# Autodesk Inventor assembly: ASY Рама №2 платформа
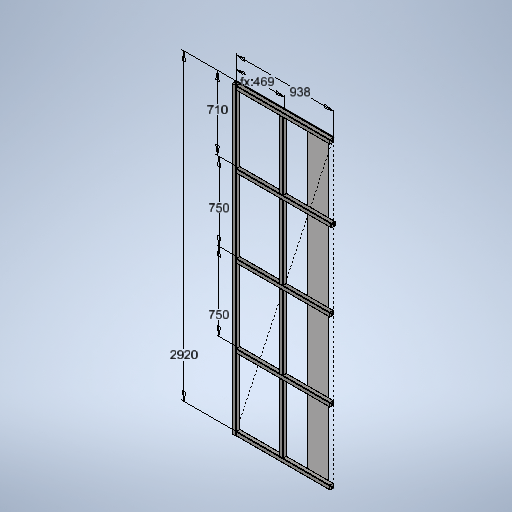
[picture p0: Inventor's stored thumbnail of the model, 512x512]
Saved by Autodesk Inventor 2025 (Build 290162010, 162A)
## iProperties
_SolveAssemblyDoc: Frame Generator Solve Assembly
_Version: 25.0.0
Created: 2025-01-19
Part Number: ASY Рама №2 платформа
Document SubType Name: Assembly
Designer: pokla
Author: pokla
## Documents named in this file (4)
- C:\Users\pokla\Documents\Inventor\NDM-VOS_powder_hopper\ASY Рама №2 платформа.iam
- C:\Users\pokla\Documents\Inventor\NDM-VOS_powder_hopper\ASY Рама №2 платформа.ipt
- C:\Users\pokla\Documents\Inventor\NDM-VOS_powder_hopper\ASY Рама №2 платформа1.ipt
- C:\Users\pokla\Documents\Inventor\NDM-VOS_powder_hopper\ASY Рама №2 платформа\Frame\Frame 1737400283119.iam
## Components (3 placed, 2 different names)
1. ASY Рама №2 платформа:1
2. ASY Рама №2 платформа:3 — Mate:1, Flush:1, Flush:2
3. Frame 1737400283119:1 [sub-assembly] — Mate:1, Flush:1, Flush:2
## Relationships (3: Flush 2, Mate 1)
- Mate:1: ASY Рама №2 платформа:3 ↔ Frame 1737400283119:1
- Flush:1: ASY Рама №2 платформа:3 ↔ Frame 1737400283119:1
- Flush:2 (50 mm): ASY Рама №2 платформа:3 ↔ Frame 1737400283119:1
